# Autodesk Inventor assembly: handle_left
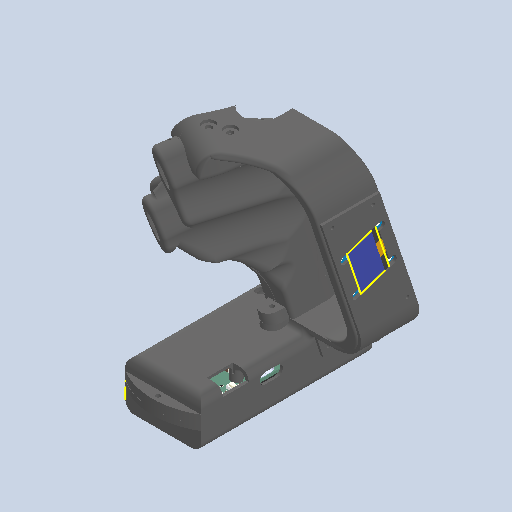
[picture p0: Inventor's stored thumbnail of the model, 512x512]
Saved by Autodesk Inventor 2026.1 (Build 301233020, 233B)
## iProperties
Created: 2026-01-22
Part Number: handle_left
Document SubType Name: Assembly
Designer: hibik
Author: hibik
## Documents named in this file (5)
- C:\Users\hibik\Documents\Robomech\HR\controller\hard\handle_left\handle_left.iam
- C:\Users\hibik\Documents\Robomech\HR\controller\hard\handle_left\handle_outside_left.ipt
- C:\Users\hibik\Documents\Robomech\HR\controller\hard\handle_left\handle_inside_left.ipt
- C:\Users\hibik\Documents\Robomech\HR\controller\hard\handle_left\handle_monitor_left.iam
- C:\Users\hibik\Documents\Robomech\HR\controller\hard\handle_left\handle_inside_cover_left.ipt
## Components (4 placed, 4 different names)
1. handle_outside_left:1 — メイト:5, メイト:6, フラッシュ:5, フラッシュ:6, フラッシュ:7
2. handle_inside_left:1 — メイト:5, メイト:6, フラッシュ:5, フラッシュ:6, フラッシュ:7
3. handle_monitor_left:1 [sub-assembly]
4. handle_inside_cover_left:1
## Relationships (5: Flush 3, Mate 2)
- メイト:5 [Mate]: handle_outside_left:1 ↔ handle_inside_left:1
- メイト:6 [Mate]: handle_outside_left:1 ↔ handle_inside_left:1
- フラッシュ:5 [Flush]: handle_outside_left:1 ↔ handle_inside_left:1
- フラッシュ:6 [Flush]: handle_outside_left:1 ↔ handle_inside_left:1
- フラッシュ:7 [Flush]: handle_outside_left:1 ↔ handle_inside_left:1
